# Autodesk Inventor assembly: ЛЦМК000002.00.04.00.02.00 2 xiao
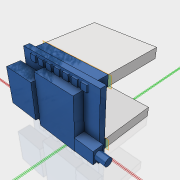
[picture p0: Inventor's stored thumbnail of the model, 180x180]
Saved by Autodesk Inventor 2021.2 (Build 252289000, 289)
## iProperties
Created: 2025-10-22
Part Number: ЛЦМК000002.00.04.00.02.00 2 xiao
Document SubType Name: Assembly
Designer: Захаров
Author: Захаров
## Documents named in this file (4)
- C:\Users\User\Documents\CaseARHead1\ЛЦМК000002.00.04.00.02.00 2 xiao.iam
- C:\Users\User\Documents\CaseARHead1\ЛЦМК.00002.00.00.00.00.01.ipt
- C:\Users\User\Documents\CaseARHead1\ЛЦМК0000002.00.00.00.00.03.ipt
- C:\Users\User\Documents\CaseARHead1\ЛЦМК.00002.00.00.00.00.21 Контакты.ipt
## Components (5 placed, 3 different names)
1. ЛЦМК.00002.00.00.00.00.01:1 — Совмещение:2, Заподлицо:3, Заподлицо:4, Заподлицо:7, Заподлицо:8, Заподлицо:9
2. ЛЦМК0000002.00.00.00.00.03:1 — Совмещение:1, Заподлицо:1, Заподлицо:2, Совмещение:2, Заподлицо:3, Заподлицо:4
3. ЛЦМК.00002.00.00.00.00.01:2 — Совмещение:1, Заподлицо:1, Заподлицо:2, Заподлицо:5, Заподлицо:6
4. ЛЦМК.00002.00.00.00.00.21 Контакты:1 — Заподлицо:5, Заподлицо:6
5. ЛЦМК.00002.00.00.00.00.21 Контакты:2 — Заподлицо:7, Заподлицо:8, Заподлицо:9
## Relationships (11: Flush 9, Mate 2)
- Совмещение:1 [Mate]: ЛЦМК0000002.00.00.00.00.03:1 ↔ ЛЦМК.00002.00.00.00.00.01:2
- Заподлицо:1 [Flush]: ЛЦМК0000002.00.00.00.00.03:1 ↔ ЛЦМК.00002.00.00.00.00.01:2
- Заподлицо:2 [Flush] (2 mm): ЛЦМК0000002.00.00.00.00.03:1 ↔ ЛЦМК.00002.00.00.00.00.01:2
- Совмещение:2 [Mate]: ЛЦМК.00002.00.00.00.00.01:1 ↔ ЛЦМК0000002.00.00.00.00.03:1
- Заподлицо:3 [Flush]: ЛЦМК.00002.00.00.00.00.01:1 ↔ ЛЦМК0000002.00.00.00.00.03:1
- Заподлицо:4 [Flush] (2 mm): ЛЦМК.00002.00.00.00.00.01:1 ↔ ЛЦМК0000002.00.00.00.00.03:1
- Заподлицо:5 [Flush]: ЛЦМК.00002.00.00.00.00.01:2 ↔ ЛЦМК.00002.00.00.00.00.21 Контакты:1
- Заподлицо:6 [Flush]: ЛЦМК.00002.00.00.00.00.01:2 ↔ ЛЦМК.00002.00.00.00.00.21 Контакты:1
- Заподлицо:7 [Flush]: ЛЦМК.00002.00.00.00.00.01:1 ↔ ЛЦМК.00002.00.00.00.00.21 Контакты:2
- Заподлицо:8 [Flush]: ЛЦМК.00002.00.00.00.00.01:1 ↔ ЛЦМК.00002.00.00.00.00.21 Контакты:2
- Заподлицо:9 [Flush]: ЛЦМК.00002.00.00.00.00.01:1 ↔ ЛЦМК.00002.00.00.00.00.21 Контакты:2
